# Autodesk Inventor assembly: Módulo Carrete-Plato correaT5
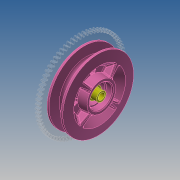
[picture p0: Inventor's stored thumbnail of the model, 180x180]
Saved by Autodesk Inventor 2017 (Build 210142000, 142)
## iProperties
Part Number: Módulo Carrete-Plato correaT5
Material: Genérico
Document SubType Name: Assembly
Designer: Leo
Author: Leo
## Documents named in this file (3)
- C:\Users\Leo\Dropbox\E\Caja Motriz\transmision Engranajes\Módulo Carrete-Plato correaT5.iam
- C:\Users\Leo\Dropbox\E\Caja Motriz\transmision Engranajes\carrete.ipt
- C:\Users\Leo\Dropbox\E\Caja Motriz\transmision Engranajes\engrane.ipt
## Components (2 placed, 2 different names)
1. carrete:1 — Insertar:1
2. engrane:1 — Insertar:1, Nivelación:1
## Relationships (2: Insert 1, Flush 1)
- Insertar:1: carrete:1 ↔ engrane:1
- Nivelación:1 [Flush]: engrane:1
